# Autodesk Inventor assembly: CNC-1.1v-XP-1-(face plate)
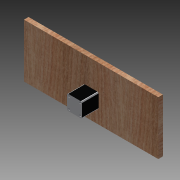
[picture p0: Inventor's stored thumbnail of the model, 180x180]
Saved by Autodesk Inventor 2015 (Build 190159000, 159)
## iProperties
Created: 2015-07-11
Part Number: CNC-1.1v-XP-1-(face plate)
Document SubType Name: Assembly
Designer: Bangladesh
Author: Bangladesh
## Documents named in this file (4)
- C:\Users\Alvi\Documents\CNC design files\CNC_1.1v\CNC-1.1v-XP-1-(face plate).iam
- C:\Users\Alvi\Documents\CNC design files\CNC_1.1v\CNC-1.1v-X-6-(end plate step.).ipt
- C:\Users\Alvi\Documents\CNC design files\CNC_1.0v\CNC- Stepper Motor.ipt
- C:\Users\Alvi\Documents\CNC design files\CNC_1.1v\CNC-1.1v-S-1-( thread coupler).ipt
## Components (3 placed, 3 different names)
1. CNC-1.1v-X-6-(end plate step.):1 — Mate:1, Mate:2, Mate:3
2. CNC- Stepper Motor:1 — Mate:1, Mate:2, Mate:3, Mate:4, Mate:5
3. CNC-1.1v-S-1-( thread coupler):1 — Mate:4, Mate:5
## Relationships (5: Mate 5)
- Mate:1: CNC-1.1v-X-6-(end plate step.):1 ↔ CNC- Stepper Motor:1
- Mate:2: CNC-1.1v-X-6-(end plate step.):1 ↔ CNC- Stepper Motor:1
- Mate:3: CNC-1.1v-X-6-(end plate step.):1 ↔ CNC- Stepper Motor:1
- Mate:4: CNC- Stepper Motor:1 ↔ CNC-1.1v-S-1-( thread coupler):1
- Mate:5: CNC- Stepper Motor:1 ↔ CNC-1.1v-S-1-( thread coupler):1
